# Autodesk Inventor assembly: dining_table
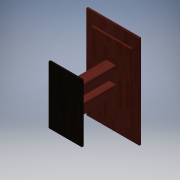
[picture p0: Inventor's stored thumbnail of the model, 180x180]
Saved by Autodesk Inventor 2019 (Build 230136000, 136)
## iProperties
Created: 2019-04-29
Part Number: dining_table
Document SubType Name: Assembly
Designer: Alex
Author: Alex
## Documents named in this file (5)
- P:\Alex\Git\3d_models\dining_table\dining_table.iam
- P:\Alex\Git\3d_models\dining_table\adapter.ipt
- P:\Alex\Git\3d_models\dining_table\stand.ipt
- P:\Alex\Git\3d_models\dining_table\tabletop.ipt
- P:\Alex\Git\3d_models\dining_table\baseplate.ipt
## Components (5 placed, 4 different names)
1. stand:1 — Flush:6, Flush:8, Mate:8
2. tabletop:1 — Flush:5, Flush:6, Flush:7, Flush:8, Mate:6, Flush:9, Flush:10, Flush:11, Flush:12
3. stand:2 — Flush:5, Flush:7, Mate:7, Mate:9
4. adapter:2 — Mate:6, Flush:9, Flush:10, Mate:7
5. baseplate:1 — Mate:8, Flush:11, Flush:12, Mate:9
## Relationships (12: Flush 8, Mate 4)
- Flush:5 (-500 mm): tabletop:1 ↔ stand:2
- Flush:6 (-500 mm): stand:1 ↔ tabletop:1
- Flush:7 (325 mm): tabletop:1 ↔ stand:2
- Flush:8 (325 mm): stand:1 ↔ tabletop:1
- Mate:6: tabletop:1 ↔ adapter:2
- Flush:9 (100 mm): tabletop:1 ↔ adapter:2
- Flush:10 (175 mm): tabletop:1 ↔ adapter:2
- Mate:7: stand:2 ↔ adapter:2
- Mate:8: stand:1 ↔ baseplate:1
- Flush:11 (150 mm): tabletop:1 ↔ baseplate:1
- Flush:12 (262.5 mm): tabletop:1 ↔ baseplate:1
- Mate:9: stand:2 ↔ baseplate:1
